# Autodesk Inventor assembly: Structure
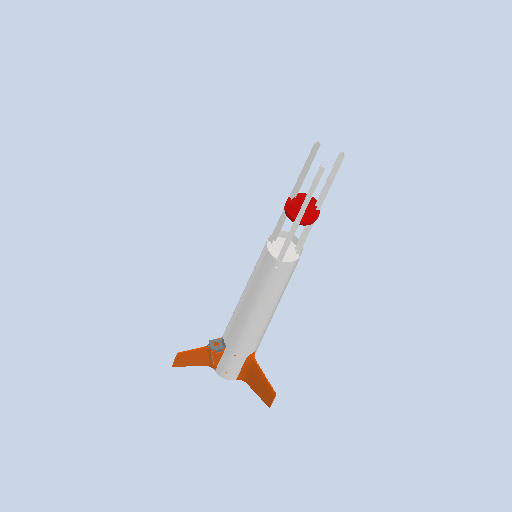
[picture p0: Inventor's stored thumbnail of the model, 512x512]
Saved by Autodesk Inventor 2024 (Build 280153000, 153)
## iProperties
Created: 2023-12-30
Part Number: Structure
Document SubType Name: Assembly
Designer: Jamie
Mass: 490.976 g
Surface Area: 3690.03 cm^2
Volume: 269.832 cm^3
Density: 1.81956 g/cm^3
Author: Jamie
## Documents named in this file (7)
- C:\Users\auror\Documents\TU Delft\DARE\Git\Scrambler-2-CAD\Autodesk\Structure.iam
- C:\Users\auror\Documents\TU Delft\DARE\Git\Scrambler-2-CAD\Autodesk\Engine bulkhead.ipt
- C:\Users\auror\Documents\TU Delft\DARE\Git\Scrambler-2-CAD\Autodesk\Stringer.ipt
- C:\Users\auror\Documents\TU Delft\DARE\Git\Scrambler-2-CAD\Autodesk\Parachute bulkhead.ipt
- C:\Users\auror\Documents\TU Delft\DARE\Git\Scrambler-2-CAD\Autodesk\Engine skin sheet metal.ipt
- C:\Users\auror\Documents\TU Delft\DARE\Git\Scrambler-2-CAD\Autodesk\Fins with camera.ipt
- C:\Users\auror\Documents\TU Delft\DARE\Git\Scrambler-2-CAD\Autodesk\Camera retention.ipt
## Components (8 placed, 6 different names)
1. Engine bulkhead:1 — Mate:32, Mate:34, Mate:37, Mate:38, Mate:39
2. Stringer:1 — Mate:12, Mate:35, Mate:37
3. Stringer:2 — Mate:13, Mate:31, Mate:33, Mate:38, Mate:39
4. Stringer:3 — Mate:11, Mate:36, Mate:40
5. Parachute bulkhead:1 — Mate:11, Mate:12, Mate:13, Mate:31, Mate:40
6. Engine skin sheet metal:1 — Mate:32, Mate:33, Mate:34, Mate:35, Mate:36, Mate:41, Mate:42
7. Fins with camera:1 — Mate:41, Mate:42, Mate:43, Mate:44, Angle:1
8. Camera retention:1 — Mate:43, Mate:44, Angle:1
## Relationships (18: Mate 17, Angle 1)
- Mate:11 (0.5 mm): Stringer:3 ↔ Parachute bulkhead:1
- Mate:12 (0.5 mm): Stringer:1 ↔ Parachute bulkhead:1
- Mate:13 (0.5 mm): Stringer:2 ↔ Parachute bulkhead:1
- Mate:31: Stringer:2 ↔ Parachute bulkhead:1
- Mate:32: Engine bulkhead:1 ↔ Engine skin sheet metal:1
- Mate:33: Stringer:2 ↔ Engine skin sheet metal:1
- Mate:34: Engine bulkhead:1 ↔ Engine skin sheet metal:1
- Mate:35: Stringer:1 ↔ Engine skin sheet metal:1
- Mate:36: Stringer:3 ↔ Engine skin sheet metal:1
- Mate:37: Engine bulkhead:1 ↔ Stringer:1
- Mate:38: Engine bulkhead:1 ↔ Stringer:2
- Mate:39: Engine bulkhead:1 ↔ Stringer:2
- Mate:40: Stringer:3 ↔ Parachute bulkhead:1
- Mate:41: Engine skin sheet metal:1 ↔ Fins with camera:1
- Mate:42: Engine skin sheet metal:1 ↔ Fins with camera:1
- Mate:43: Fins with camera:1 ↔ Camera retention:1
- Mate:44: Fins with camera:1 ↔ Camera retention:1
- Angle:1 (90 deg): Fins with camera:1 ↔ Camera retention:1
